# Autodesk Inventor assembly: Zespół1
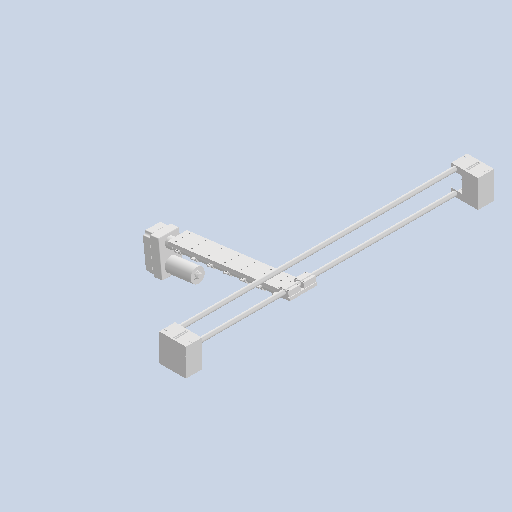
[picture p0: Inventor's stored thumbnail of the model, 512x512]
Saved by Autodesk Inventor 2025.2 (Build 292293000, 293)
## iProperties
Created: 2025-03-20
Part Number: Zespół1
Document SubType Name: Assembly
Designer: rango
Author: rango
## Documents named in this file (9)
- C:\Users\tadek\Documents\Inventor_projekt_inzynierski\Zespół1.iam
- C:\Users\tadek\Documents\Inventor_projekt_inzynierski\walek_liniowy_fi16_L1000.ipt
- C:\Users\tadek\Documents\Inventor_projekt_inzynierski\lozysko_liniowe_44L_35W_20H_fi16.ipt
- C:\Users\tadek\Documents\Inventor_projekt_inzynierski\plaskownik_uchwyt_silownika_L460_W100_H10.ipt
- C:\Users\tadek\Documents\Inventor_projekt_inzynierski\silownik_L556_H125_W75_A300.ipt
- C:\Users\tadek\Documents\Inventor_projekt_inzynierski\obejma_fi32_L44.ipt
- C:\Users\tadek\Documents\Inventor_projekt_inzynierski\obudowa_silnik_H100_L11_W56.ipt
- C:\Users\tadek\Documents\Inventor_projekt_inzynierski\silnik_krokowy_W56.4xH56.4xL56.ipt
- C:\Users\tadek\Documents\Inventor_projekt_inzynierski\kolo_zebate_do_pasa_fi32_6,370_L19.ipt
## Components (26 placed, 8 different names)
1. walek_liniowy_fi16_L1000:1 — Zestawiające:1, Zestawiające:2, Wstawiające:28, Wstawiające:29
2. lozysko_liniowe_44L_35W_20H_fi16:1 — Zestawiające:1, Zestawiające:6
3. lozysko_liniowe_44L_35W_20H_fi16:2 — Zestawiające:2, Wstawiające:27
4. plaskownik_uchwyt_silownika_L460_W100_H10:1 — Wstawiające:5, Wstawiające:6, Wstawiające:7, Wstawiające:8, Wstawiające:9, Wstawiające:10, Wstawiające:11, Wstawiające:27, Zestawiające:6, Zestawiające:14
5. silownik_L556_H125_W75_A300:1 — Wstawiające:26, Zestawiające:5, Zestawiające:7, Kątowe:1, Kątowe:2, Kątowe:3, Kątowe:4, Kątowe:5
6. obejma_fi32_L44:1 — Wstawiające:6, Wstawiające:14, Wstawiające:15, Zestawiające:7, Kątowe:1
7. obejma_fi32_L44:2 — Wstawiające:5, Wstawiające:12, Wstawiające:13, Wstawiające:26
8. obejma_fi32_L44:3 — Wstawiające:7, Wstawiające:16, Wstawiające:17
9. obejma_fi32_L44:4 — Wstawiające:8, Wstawiające:18, Wstawiające:19
10. obejma_fi32_L44:5 — Wstawiające:9, Wstawiające:20, Wstawiające:21
11. obejma_fi32_L44:6 — Wstawiające:10, Wstawiające:22, Wstawiające:23
12. obejma_fi32_L44:7 — Wstawiające:11, Wstawiające:24, Wstawiające:25, Zestawiające:5
13. obejma_fi32_L44:8 — Wstawiające:12, Wstawiające:13
14. obejma_fi32_L44:9 — Wstawiające:14, Wstawiające:15
15. obejma_fi32_L44:10 — Wstawiające:16, Wstawiające:17, Kątowe:2
16. obejma_fi32_L44:11 — Wstawiające:18, Wstawiające:19, Kątowe:3
17. obejma_fi32_L44:12 — Wstawiające:20, Wstawiające:21, Kątowe:4
18. obejma_fi32_L44:13 — Wstawiające:22, Wstawiające:23, Kątowe:5
19. obejma_fi32_L44:14 — Wstawiające:24, Wstawiające:25
20. obudowa_silnik_H100_L11_W56:1 — Wstawiające:28, Wstawiające:31, Zestawiające:8, Zestawiające:12, Zestawiające:13
21. obudowa_silnik_H100_L11_W56:2 — Wstawiające:29, Wstawiające:30, Zestawiające:9, Zestawiające:10, Zestawiające:11
22. walek_liniowy_fi16_L1000:2 — Wstawiające:30, Wstawiające:31
23. silnik_krokowy_W56.4xH56.4xL56:1 — Zestawiające:9, Zestawiające:10, Zestawiające:11, Wstawiające:33
24. silnik_krokowy_W56.4xH56.4xL56:2 — Zestawiające:8, Zestawiające:12, Zestawiające:13, Wstawiające:32
25. kolo_zebate_do_pasa_fi32_6,370_L19:1 — Wstawiające:32
26. kolo_zebate_do_pasa_fi32_6,370_L19:2 — Wstawiające:33
## Relationships (46: Insert 29, Mate 12, Angle 5)
- Zestawiające:1 [Mate]: walek_liniowy_fi16_L1000:1 ↔ lozysko_liniowe_44L_35W_20H_fi16:1
- Zestawiające:2 [Mate]: walek_liniowy_fi16_L1000:1 ↔ lozysko_liniowe_44L_35W_20H_fi16:2
- Wstawiające:5 [Insert]: plaskownik_uchwyt_silownika_L460_W100_H10:1 ↔ obejma_fi32_L44:2
- Wstawiające:6 [Insert]: plaskownik_uchwyt_silownika_L460_W100_H10:1 ↔ obejma_fi32_L44:1
- Wstawiające:7 [Insert]: plaskownik_uchwyt_silownika_L460_W100_H10:1 ↔ obejma_fi32_L44:3
- Wstawiające:8 [Insert]: plaskownik_uchwyt_silownika_L460_W100_H10:1 ↔ obejma_fi32_L44:4
- Wstawiające:9 [Insert]: plaskownik_uchwyt_silownika_L460_W100_H10:1 ↔ obejma_fi32_L44:5
- Wstawiające:10 [Insert]: plaskownik_uchwyt_silownika_L460_W100_H10:1 ↔ obejma_fi32_L44:6
- Wstawiające:11 [Insert]: plaskownik_uchwyt_silownika_L460_W100_H10:1 ↔ obejma_fi32_L44:7
- Wstawiające:12 [Insert]: obejma_fi32_L44:2 ↔ obejma_fi32_L44:8
- Wstawiające:13 [Insert]: obejma_fi32_L44:2 ↔ obejma_fi32_L44:8
- Wstawiające:14 [Insert]: obejma_fi32_L44:1 ↔ obejma_fi32_L44:9
- Wstawiające:15 [Insert]: obejma_fi32_L44:1 ↔ obejma_fi32_L44:9
- Wstawiające:16 [Insert]: obejma_fi32_L44:3 ↔ obejma_fi32_L44:10
- Wstawiające:17 [Insert]: obejma_fi32_L44:3 ↔ obejma_fi32_L44:10
- Wstawiające:18 [Insert]: obejma_fi32_L44:4 ↔ obejma_fi32_L44:11
- Wstawiające:19 [Insert]: obejma_fi32_L44:4 ↔ obejma_fi32_L44:11
- Wstawiające:20 [Insert]: obejma_fi32_L44:5 ↔ obejma_fi32_L44:12
- Wstawiające:21 [Insert]: obejma_fi32_L44:5 ↔ obejma_fi32_L44:12
- Wstawiające:22 [Insert]: obejma_fi32_L44:6 ↔ obejma_fi32_L44:13
- Wstawiające:23 [Insert]: obejma_fi32_L44:6 ↔ obejma_fi32_L44:13
- Wstawiające:24 [Insert]: obejma_fi32_L44:7 ↔ obejma_fi32_L44:14
- Wstawiające:25 [Insert]: obejma_fi32_L44:7 ↔ obejma_fi32_L44:14
- Wstawiające:26 [Insert]: silownik_L556_H125_W75_A300:1 ↔ obejma_fi32_L44:2
- Zestawiające:5 [Mate]: silownik_L556_H125_W75_A300:1 ↔ obejma_fi32_L44:7
- Wstawiające:27 [Insert]: lozysko_liniowe_44L_35W_20H_fi16:2 ↔ plaskownik_uchwyt_silownika_L460_W100_H10:1
- Zestawiające:6 [Mate]: lozysko_liniowe_44L_35W_20H_fi16:1 ↔ plaskownik_uchwyt_silownika_L460_W100_H10:1
- Zestawiające:7 [Mate]: silownik_L556_H125_W75_A300:1 ↔ obejma_fi32_L44:1
- Kątowe:1 [Angle] (0 deg): silownik_L556_H125_W75_A300:1 ↔ obejma_fi32_L44:1
- Kątowe:2 [Angle] (0 deg): silownik_L556_H125_W75_A300:1 ↔ obejma_fi32_L44:10
- Kątowe:3 [Angle] (0 deg): silownik_L556_H125_W75_A300:1 ↔ obejma_fi32_L44:11
- Kątowe:4 [Angle] (0 deg): silownik_L556_H125_W75_A300:1 ↔ obejma_fi32_L44:12
- Kątowe:5 [Angle] (0 deg): silownik_L556_H125_W75_A300:1 ↔ obejma_fi32_L44:13
- Wstawiające:28 [Insert]: walek_liniowy_fi16_L1000:1 ↔ obudowa_silnik_H100_L11_W56:1
- Wstawiające:29 [Insert]: walek_liniowy_fi16_L1000:1 ↔ obudowa_silnik_H100_L11_W56:2
- Wstawiające:30 [Insert]: obudowa_silnik_H100_L11_W56:2 ↔ walek_liniowy_fi16_L1000:2
- Wstawiające:31 [Insert]: obudowa_silnik_H100_L11_W56:1 ↔ walek_liniowy_fi16_L1000:2
- Zestawiające:8 [Mate]: obudowa_silnik_H100_L11_W56:1 ↔ silnik_krokowy_W56.4xH56.4xL56:2
- Zestawiające:9 [Mate]: obudowa_silnik_H100_L11_W56:2 ↔ silnik_krokowy_W56.4xH56.4xL56:1
- Zestawiające:10 [Mate]: obudowa_silnik_H100_L11_W56:2 ↔ silnik_krokowy_W56.4xH56.4xL56:1
- Zestawiające:11 [Mate]: obudowa_silnik_H100_L11_W56:2 ↔ silnik_krokowy_W56.4xH56.4xL56:1
- Zestawiające:12 [Mate]: obudowa_silnik_H100_L11_W56:1 ↔ silnik_krokowy_W56.4xH56.4xL56:2
- Zestawiające:13 [Mate]: obudowa_silnik_H100_L11_W56:1 ↔ silnik_krokowy_W56.4xH56.4xL56:2
- Wstawiające:32 [Insert]: silnik_krokowy_W56.4xH56.4xL56:2 ↔ kolo_zebate_do_pasa_fi32_6,370_L19:1
- Wstawiające:33 [Insert]: silnik_krokowy_W56.4xH56.4xL56:1 ↔ kolo_zebate_do_pasa_fi32_6,370_L19:2
- Zestawiające:14 [Mate]: plaskownik_uchwyt_silownika_L460_W100_H10:1
